# Autodesk Inventor assembly: Support bobine
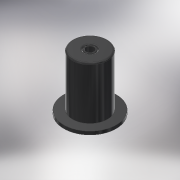
[picture p0: Inventor's stored thumbnail of the model, 180x180]
Saved by Autodesk Inventor 2017 (Build 210142000, 142)
## iProperties
Company: FABLAB Frenchmakers
Part Number: Support bobine
Material: Générique
Document SubType Name: Assembly
Designer: FABLAB Frenchmakers
Mass: 198.228 g
Surface Area: 505.096 cm^2
Volume: 176.708 cm^3
Density: 1.12178 g/cm^3
Project: 1420 Vauban 3D XL
Catalog Web Link: http://frenchmakers.com/
Stock Number: 1420-03-00
## Documents named in this file (6)
- W:\Professionnel\Conception FABLAB\1420-Vauban 3D XL\1420-03 Support bobine filament\1420-03-00 Support bobine.iam
- W:\Professionnel\Conception FABLAB\1420-Vauban 3D XL\1420-03 Support bobine filament\1420-03-02 Support.ipt
- W:\Professionnel\Conception FABLAB\1420-Vauban 3D XL\1420-03 Support bobine filament\1420-03-04 Roulement a bille 608ZZ.ipt
- W:\Professionnel\Conception FABLAB\1420-Vauban 3D XL\1420-03 Support bobine filament\1420-03-03 Adapteur.ipt
- W:\Professionnel\Conception FABLAB\1420-Vauban 3D XL\1420-03 Support bobine filament\1420-03-01 Entretoise.ipt
- W:\Professionnel\Conception FABLAB\1420-Vauban 3D XL\1420-90 Centre de contenu\fr-FR\ANSI B18.3.1M(1)\ANSI B18.3.1M - M5x0,8 x 30(2).ipt
## Components (5 placed, 5 different names)
1. 1420-03-02 Support:1 — Placage:2, Placage:3, Placage:5, Placage:6, Logement:2
2. 1420-03-04 Roulement a bille 608ZZ:1 — Placage:2, Placage:3, Logement:1
3. 1420-03-03 Adapteur:1 — Placage:5, Placage:6
4. 1420-03-01 Entretoise:1 — Logement:1
5. Vis à tête percée - Métrique M5x0,8 x 30:1 — Logement:2
## Relationships (6: Mate 4, Insert 2)
- Placage:2 [Mate]: 1420-03-02 Support:1 ↔ 1420-03-04 Roulement a bille 608ZZ:1
- Placage:3 [Mate]: 1420-03-02 Support:1 ↔ 1420-03-04 Roulement a bille 608ZZ:1
- Placage:5 [Mate]: 1420-03-02 Support:1 ↔ 1420-03-03 Adapteur:1
- Placage:6 [Mate]: 1420-03-02 Support:1 ↔ 1420-03-03 Adapteur:1
- Logement:1 [Insert]: 1420-03-04 Roulement a bille 608ZZ:1 ↔ 1420-03-01 Entretoise:1
- Logement:2 [Insert]: 1420-03-02 Support:1 ↔ Vis à tête percée - Métrique M5x0,8 x 30:1
